# Autodesk Inventor assembly: Assembly1
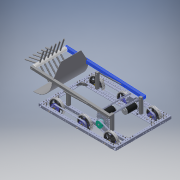
[picture p0: Inventor's stored thumbnail of the model, 180x180]
Saved by Autodesk Inventor 2016 (Build 200138000, 138)
## iProperties
Created: 2016-09-04
Part Number: Assembly1
Document SubType Name: Assembly
Designer: gus
Author: gus
## Documents named in this file (16)
- \\Mac\Home\Desktop\bunnybots 2016\prototype\Assembly1.iam
- \\Mac\Home\Desktop\bunnybots 2016\prototype\C-Base2LongTBMini6HiGripBelts.iam
- \\Mac\Home\Desktop\bunnybots 2016\prototype\Part88.ipt
- \\Mac\Home\Desktop\bunnybots 2016\prototype\Part89.ipt
- \\Mac\Home\Desktop\bunnybots 2016\prototype\Part90.ipt
- \\Mac\Home\Desktop\bunnybots 2016\prototype\Part88_MIR.ipt
- \\Mac\Home\Desktop\bunnybots 2016\prototype\Part89_MIR.ipt
- \\Mac\Home\Desktop\bunnybots 2016\prototype\Part93.ipt
- \\Mac\Home\Desktop\bunnybots 2016\prototype\Part95.ipt
- \\Mac\Home\Desktop\bunnybots 2016\prototype\Part1.ipt
- \\Mac\Home\Desktop\bunnybots 2016\prototype\Part2.ipt
- \\Mac\Home\Desktop\bunnybots 2016\prototype\Part3.ipt
- \\Mac\Home\Desktop\bunnybots 2016\prototype\Part1_MIR.ipt
- \\Mac\Home\Desktop\bunnybots 2016\prototype\Part2_MIR.ipt
- \\Mac\Home\Desktop\bunnybots 2016\prototype\Part3_MIR.ipt
- \\Mac\Home\Desktop\bunnybots 2016\prototype\Part7.ipt
## Components (32 placed, 15 different names)
1. C-Base2LongTBMini6HiGripBelts:1 [sub-assembly] — Flush:4, Mate:2, Mate:3, Mate:5, Flush:7, Flush:8, Mate:8, Tangent:2, Flush:14, Flush:15, Flush:18
2. Part88:2 — Flush:4, Mate:2, Flush:5, Cylindrical:1, Mate:3, Mate:5, Flush:9
3. Part89:1 — Flush:5, Cylindrical:1, Flush:6, Mate:4, Mate:6, Cylindrical:10
4. Part90:1 — Flush:6, Mate:4, Mate:6, Mate:9, Flush:19
5. Part88_MIR:1 — Mate:7, Cylindrical:2, Flush:8, Flush:9, Mate:8, Mate:12
6. Part89_MIR:1 — Mate:7, Cylindrical:2, Mate:9, Flush:10, Cylindrical:3, Cylindrical:7
7. Part93:1 — Flush:10, Cylindrical:3, Mate:10, Mate:11, Tangent:1
8. Part1:1 — Cylindrical:4, Tangent:2, Cylindrical:6
9. Part2:1 — Cylindrical:4, Cylindrical:7
10. Part3:1 — Flush:14, Flush:15, Cylindrical:6, Mate:12, Flush:16, Flush:17
11. Part1_MIR:1 — Cylindrical:8, Cylindrical:9, Tangent:3
12. Part2_MIR:1 — Cylindrical:8, Cylindrical:10
13. Part3_MIR:1 — Cylindrical:9, Flush:16, Flush:17, Flush:18, Tangent:3
14. Part7:1 — Flush:19
15. Part95:1 — Mate:10, Mate:11, Tangent:1
16. Part95:2
17. Part95:3
18. Part95:4
19. Part95:5
20. Part95:6
21. Part95:7
22. Part95:8
23. Part95:9
24. Part95:10
25. Part95:11
26. Part95:12
27. Part95:13
28. Part95:14
29. Part95:15
30. Part95:16
31. Part95:17
32. Part95:18
## Component patterns: (3 elements), (6 elements, first: Part95:1), Component Pattern 1:2 (6 elements), Component Pattern 1:3 (6 elements)
## Relationships (36: Flush 13, Mate 11, CylindricalJoint 9, Tangent 3)
- Flush:4: C-Base2LongTBMini6HiGripBelts:1 ↔ Part88:2
- Mate:2: C-Base2LongTBMini6HiGripBelts:1 ↔ Part88:2
- Flush:5: Part88:2 ↔ Part89:1
- Cylindrical:1: Part88:2 ↔ Part89:1
- Mate:3: C-Base2LongTBMini6HiGripBelts:1 ↔ Part88:2
- Flush:6: Part89:1 ↔ Part90:1
- Mate:4: Part89:1 ↔ Part90:1
- Mate:5: C-Base2LongTBMini6HiGripBelts:1 ↔ Part88:2
- Mate:6 (-228.6 mm): Part89:1 ↔ Part90:1
- Flush:7 (-292.1 mm): C-Base2LongTBMini6HiGripBelts:1
- Mate:7: Part88_MIR:1 ↔ Part89_MIR:1
- Cylindrical:2: Part88_MIR:1 ↔ Part89_MIR:1
- Flush:8: C-Base2LongTBMini6HiGripBelts:1 ↔ Part88_MIR:1
- Flush:9: Part88:2 ↔ Part88_MIR:1
- Mate:8: C-Base2LongTBMini6HiGripBelts:1 ↔ Part88_MIR:1
- Mate:9: Part90:1 ↔ Part89_MIR:1
- Flush:10: Part89_MIR:1 ↔ Part93:1
- Cylindrical:3: Part89_MIR:1 ↔ Part93:1
- Mate:10: Part93:1 ↔ Part95:1
- Mate:11: Part93:1 ↔ Part95:1
- Tangent:1 (50.8 mm): Part93:1 ↔ Part95:1
- Cylindrical:4: Part1:1 ↔ Part2:1
- Tangent:2: C-Base2LongTBMini6HiGripBelts:1 ↔ Part1:1
- Flush:14: C-Base2LongTBMini6HiGripBelts:1 ↔ Part3:1
- Flush:15: C-Base2LongTBMini6HiGripBelts:1 ↔ Part3:1
- Cylindrical:6: Part1:1 ↔ Part3:1
- Cylindrical:7: Part89_MIR:1 ↔ Part2:1
- Mate:12 (434.7718 mm): Part88_MIR:1 ↔ Part3:1
- Cylindrical:8: Part1_MIR:1 ↔ Part2_MIR:1
- Cylindrical:9: Part1_MIR:1 ↔ Part3_MIR:1
- Flush:16: Part3:1 ↔ Part3_MIR:1
- Flush:17: Part3:1 ↔ Part3_MIR:1
- Flush:18: C-Base2LongTBMini6HiGripBelts:1 ↔ Part3_MIR:1
- Tangent:3: Part1_MIR:1 ↔ Part3_MIR:1
- Cylindrical:10: Part89:1 ↔ Part2_MIR:1
- Flush:19: Part90:1 ↔ Part7:1
